# Autodesk Inventor assembly: ETL Module Carrier V1
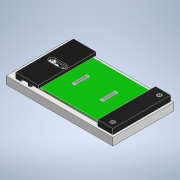
[picture p0: Inventor's stored thumbnail of the model, 180x180]
Saved by Autodesk Inventor 2022 (Build 260153000, 153)
## iProperties
Created: 2022-04-14
Part Number: ETL Module Carrier V1
Document SubType Name: Assembly
Designer: Caleb
Author: Caleb
## Documents named in this file (7)
- C:\Users\Caleb\Desktop\nebraska-silicon-lab\Hardware\ETL\Module Carrier\Module Carrier V1\ETL Module Carrier V1.iam
- C:\Users\Caleb\Desktop\nebraska-silicon-lab\Hardware\ETL\modules\tamale v1.3\Tamale - v1p3.iam
- C:\Users\Caleb\Desktop\nebraska-silicon-lab\Hardware\ETL\Module Carrier\Module Carrier V1\Carrier Plate V1.ipt
- C:\Users\Caleb\Desktop\nebraska-silicon-lab\Hardware\ETL\Module Carrier\Module Carrier V1\Carrier Clip V1.ipt
- C:\Users\Caleb\Desktop\nebraska-silicon-lab\Hardware\ETL\Module Carrier\Module Carrier V1\Holder V1.ipt
- C:\Users\Caleb\Desktop\nebraska-silicon-lab\Hardware\ETL\Module Carrier\Module Carrier V1\91771A066_Passivated 18-8 Stainless Steel Phillips Flat Head Screw.ipt
- C:\Users\Caleb\Desktop\nebraska-silicon-lab\Hardware\ETL\Module Carrier\Module Carrier V1\91770A073_Extra-Wide Truss Head Phillips Screws.ipt
## Components (7 placed, 6 different names)
1. Carrier Plate V1:1 — Mate:1, Angle:1, Mate:2, Angle:2, Mate:5, Angle:3, Insert:1, Insert:4
2. Carrier Clip V1:1 — Mate:2, Angle:2
3. 91771A066_Passivated 18-8 Stainless Steel Phillips Flat Head Screw:2 — Insert:3
4. 91771A066_Passivated 18-8 Stainless Steel Phillips Flat Head Screw:1 — Insert:2
5. Holder V1:1 — Mate:5, Angle:3, Insert:1, Insert:2, Insert:3
6. Tamale - v1p3:1 [sub-assembly] — Mate:1, Angle:1
7. 91770A073_Extra-Wide Truss Head Phillips Screws:1 — Insert:4
## Relationships (10: Insert 4, Mate 3, Angle 3)
- Mate:1: Carrier Plate V1:1 ↔ Tamale - v1p3:1
- Angle:1 (0 deg): Carrier Plate V1:1 ↔ Tamale - v1p3:1
- Mate:2: Carrier Plate V1:1 ↔ Carrier Clip V1:1
- Angle:2 (0 deg): Carrier Plate V1:1 ↔ Carrier Clip V1:1
- Mate:5: Carrier Plate V1:1 ↔ Holder V1:1
- Angle:3 (0 deg): Carrier Plate V1:1 ↔ Holder V1:1
- Insert:1: Carrier Plate V1:1 ↔ Holder V1:1
- Insert:2: 91771A066_Passivated 18-8 Stainless Steel Phillips Flat Head Screw:1 ↔ Holder V1:1
- Insert:3: 91771A066_Passivated 18-8 Stainless Steel Phillips Flat Head Screw:2 ↔ Holder V1:1
- Insert:4 (3.5052 mm): Carrier Plate V1:1 ↔ 91770A073_Extra-Wide Truss Head Phillips Screws:1
